# Autodesk Inventor assembly: FinalDT
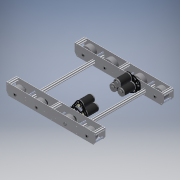
[picture p0: Inventor's stored thumbnail of the model, 180x180]
Saved by Autodesk Inventor 2016 (Build 200138000, 138)
## iProperties
Created: 2017-01-28
Part Number: FinalDT
Document SubType Name: Assembly
Designer: hamblettk
Author: hamblettk
## Documents named in this file (9)
- E:\1073CAD\Robot2017\DriveTrain\Let's try this again\FinalDT.iam
- E:\1073CAD\Robot2017\DriveTrain\Let's try this again\OutsidePlate2.ipt
- E:\1073CAD\Robot2017\DriveTrain\Individual Parts\3.625Churro.ipt
- E:\1073CAD\Robot2017\DriveTrain\Individual Parts\Mock 8020 3.375in.ipt
- E:\1073CAD\Robot2017\DriveTrain\Let's try this again\InsidePlate2.ipt
- E:\1073CAD\Robot2017\DriveTrain\Individual Parts\SinglePulley.iam
- E:\1073CAD\Robot2017\DriveTrain\Individual Parts\DoublePulleyGearbox.iam
- E:\1073CAD\Robot2017\DriveTrain\Individual Parts\DoublePulley.iam
- E:\1073CAD\Robot2017\DriveTrain\Individual Parts\Mock 8020 28.25in.ipt
## Components (38 placed, 8 different names)
1. OutsidePlate2:1 — Mate:1, Mate:2, Mate:3, Mate:4, Mate:5, Mate:7, Mate:8, Mate:9, Mate:10, Mate:11, Flush:1, Flush:2, Mate:12, Flush:3, Flush:4, Flush:5, Flush:6, Insert:1, Insert:2, Insert:3, Insert:4, Mate:15, Flush:7, Mate:17, Mate:18
2. 3.625Churro:1 — Mate:10
3. 3.625Churro:2 — Mate:8
4. 3.625Churro:3 — Mate:9
5. 3.625Churro:4 — Mate:4
6. 3.625Churro:6 — Mate:7
7. 3.625Churro:7 — Mate:5
8. 3.625Churro:8 — Mate:2
9. 3.625Churro:9 — Mate:3
10. 3.625Churro:10 — Mate:1
11. Mock 8020 3.375in:1 — Mate:11, Flush:1, Flush:2
12. Mock 8020 3.375in:2 — Mate:12, Flush:3, Flush:4, Mate:13
13. InsidePlate2:1 — Flush:5, Flush:6, Mate:13, Mate:14, Mate:16, Flush:8, Flush:9
14. SinglePulley:1 [sub-assembly] — Insert:1
15. SinglePulley:2 [sub-assembly] — Insert:2
16. DoublePulleyGearbox:1 [sub-assembly] — Insert:3, Mate:14
17. DoublePulley:1 [sub-assembly] — Insert:4
18. Mock 8020 3.375in:3 — Mate:15, Flush:7, Mate:16
19. Mock 8020 28.25in:1 — Mate:18, Mate:19
20. Mock 8020 28.25in:2 — Mate:17
21. InsidePlate2:2 — Flush:8, Flush:9, Flush:10, Flush:11, Mate:33, Mate:34
22. OutsidePlate2:2 — Flush:10, Flush:11, Mate:19, Mate:20, Mate:21, Mate:22, Mate:23, Mate:24, Mate:25, Mate:26, Mate:27, Mate:28, Mate:29, Flush:12, Flush:13, Mate:30, Flush:14, Mate:31, Flush:15, Flush:16, Mate:32, Insert:5, Insert:6, Insert:7, Insert:8
23. 3.625Churro:11 — Mate:20
24. 3.625Churro:12 — Mate:22
25. 3.625Churro:13 — Mate:21
26. 3.625Churro:14 — Mate:23
27. 3.625Churro:15 — Mate:24
28. 3.625Churro:16 — Mate:25
29. 3.625Churro:17 — Mate:26
30. 3.625Churro:18 — Mate:27
31. 3.625Churro:19 — Mate:28
32. Mock 8020 3.375in:4 — Mate:31, Flush:15, Flush:16
33. Mock 8020 3.375in:5 — Mate:30, Flush:14, Mate:32
34. Mock 8020 3.375in:6 — Mate:29, Flush:12, Flush:13, Mate:33
35. SinglePulley:3 [sub-assembly] — Insert:6
36. SinglePulley:4 [sub-assembly] — Insert:5
37. DoublePulleyGearbox:2 [sub-assembly] — Insert:7, Mate:34
38. DoublePulley:2 [sub-assembly] — Insert:8
## Relationships (57: Mate 33, Flush 16, Insert 8)
- Mate:1: OutsidePlate2:1 ↔ 3.625Churro:10
- Mate:2: OutsidePlate2:1 ↔ 3.625Churro:8
- Mate:3: OutsidePlate2:1 ↔ 3.625Churro:9
- Mate:4: OutsidePlate2:1 ↔ 3.625Churro:4
- Mate:5: OutsidePlate2:1 ↔ 3.625Churro:7
- Mate:7: OutsidePlate2:1 ↔ 3.625Churro:6
- Mate:8: OutsidePlate2:1 ↔ 3.625Churro:2
- Mate:9: OutsidePlate2:1 ↔ 3.625Churro:3
- Mate:10: OutsidePlate2:1 ↔ 3.625Churro:1
- Mate:11: OutsidePlate2:1 ↔ Mock 8020 3.375in:1
- Flush:1: OutsidePlate2:1 ↔ Mock 8020 3.375in:1
- Flush:2: OutsidePlate2:1 ↔ Mock 8020 3.375in:1
- Mate:12: OutsidePlate2:1 ↔ Mock 8020 3.375in:2
- Flush:3: OutsidePlate2:1 ↔ Mock 8020 3.375in:2
- Flush:4: OutsidePlate2:1 ↔ Mock 8020 3.375in:2
- Flush:5: OutsidePlate2:1 ↔ InsidePlate2:1
- Flush:6: OutsidePlate2:1 ↔ InsidePlate2:1
- Mate:13: Mock 8020 3.375in:2 ↔ InsidePlate2:1
- Insert:1: OutsidePlate2:1 ↔ SinglePulley:1
- Insert:2: OutsidePlate2:1 ↔ SinglePulley:2
- Insert:3: OutsidePlate2:1 ↔ DoublePulleyGearbox:1
- Mate:14: InsidePlate2:1 ↔ DoublePulleyGearbox:1
- Insert:4: OutsidePlate2:1 ↔ DoublePulley:1
- Mate:15: OutsidePlate2:1 ↔ Mock 8020 3.375in:3
- Flush:7: OutsidePlate2:1 ↔ Mock 8020 3.375in:3
- Mate:16: InsidePlate2:1 ↔ Mock 8020 3.375in:3
- Mate:17: OutsidePlate2:1 ↔ Mock 8020 28.25in:2
- Mate:18: OutsidePlate2:1 ↔ Mock 8020 28.25in:1
- Flush:8: InsidePlate2:1 ↔ InsidePlate2:2
- Flush:9: InsidePlate2:1 ↔ InsidePlate2:2
- Flush:10: InsidePlate2:2 ↔ OutsidePlate2:2
- Flush:11: InsidePlate2:2 ↔ OutsidePlate2:2
- Mate:19: Mock 8020 28.25in:1 ↔ OutsidePlate2:2
- Mate:20: OutsidePlate2:2 ↔ 3.625Churro:11
- Mate:21: OutsidePlate2:2 ↔ 3.625Churro:13
- Mate:22: OutsidePlate2:2 ↔ 3.625Churro:12
- Mate:23: OutsidePlate2:2 ↔ 3.625Churro:14
- Mate:24: OutsidePlate2:2 ↔ 3.625Churro:15
- Mate:25: OutsidePlate2:2 ↔ 3.625Churro:16
- Mate:26: OutsidePlate2:2 ↔ 3.625Churro:17
- Mate:27: OutsidePlate2:2 ↔ 3.625Churro:18
- Mate:28: OutsidePlate2:2 ↔ 3.625Churro:19
- Mate:29: OutsidePlate2:2 ↔ Mock 8020 3.375in:6
- Flush:12: OutsidePlate2:2 ↔ Mock 8020 3.375in:6
- Flush:13: OutsidePlate2:2 ↔ Mock 8020 3.375in:6
- Mate:30: OutsidePlate2:2 ↔ Mock 8020 3.375in:5
- Flush:14: OutsidePlate2:2 ↔ Mock 8020 3.375in:5
- Mate:31: OutsidePlate2:2 ↔ Mock 8020 3.375in:4
- Flush:15: OutsidePlate2:2 ↔ Mock 8020 3.375in:4
- Flush:16: OutsidePlate2:2 ↔ Mock 8020 3.375in:4
- Mate:32: OutsidePlate2:2 ↔ Mock 8020 3.375in:5
- Mate:33: InsidePlate2:2 ↔ Mock 8020 3.375in:6
- Insert:5: OutsidePlate2:2 ↔ SinglePulley:4
- Insert:6: OutsidePlate2:2 ↔ SinglePulley:3
- Insert:7: OutsidePlate2:2 ↔ DoublePulleyGearbox:2
- Mate:34: InsidePlate2:2 ↔ DoublePulleyGearbox:2
- Insert:8: OutsidePlate2:2 ↔ DoublePulley:2
